# Autodesk Inventor assembly: ktoe
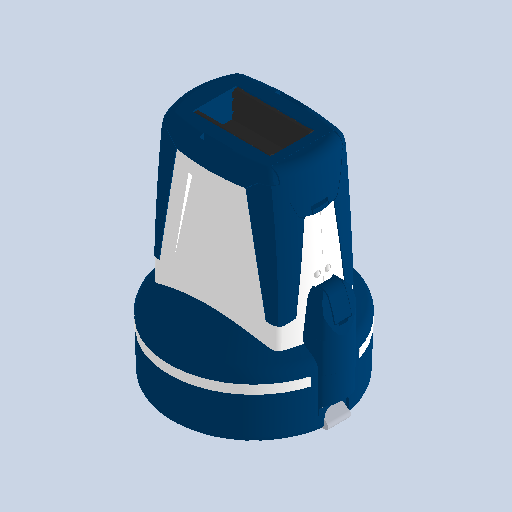
[picture p0: Inventor's stored thumbnail of the model, 512x512]
Saved by Autodesk Inventor 2023 (Build 270158000, 158)
## iProperties
Created: 2022-09-14
Part Number: ktoe
Document SubType Name: Assembly
Designer: Robert
Author: Robert
## Documents named in this file (7)
- C:\Users\Rober\Documents\Ingenieurinformatik\grop\catkin\src\grop\coactegpc\urdf\40\base\ktoe\ktoe.iam
- C:\Users\Rober\Documents\Ingenieurinformatik\grop\catkin\src\grop\coactegpc\urdf\40\base\ktoe\Co-act EGP-C 40 Modell 1.ipt
- C:\Users\Rober\Documents\Ingenieurinformatik\grop\catkin\src\grop\coactegpc\urdf\40\base\ktoe\SCHUNK-1013180-ISO-1-50-M6 Universalflansch Co-act-EGP-C.ipt
- C:\Users\Rober\Documents\Ingenieurinformatik\grop\catkin\src\grop\coactegpc\urdf\40\base\ktoe\SCHUNK-9905502 Typenschild 9x24x0_3.ipt
- C:\Users\Rober\Documents\Ingenieurinformatik\grop\catkin\src\grop\coactegpc\urdf\40\base\ktoe\SCHUNK-5521120 Gehaeuse EGP 40.ipt
- C:\Users\Rober\Documents\Ingenieurinformatik\grop\catkin\src\grop\coactegpc\urdf\40\base\ktoe\SCHUNK-SNT016581 Stecker EGP.ipt
- C:\Users\Rober\Documents\Ingenieurinformatik\grop\catkin\src\grop\coactegpc\urdf\40\base\ktoe\SCHUNK-9700901 Halter fuer NHS Du 4.ipt
## Components (8 placed, 6 different names)
1. Co-act EGP-C 40 Modell 1:1
2. SCHUNK-1013180-ISO-1-50-M6 Universalflansch Co-act-EGP-C:1
3. SCHUNK-9905502 Typenschild 9x24x0_3:1
4. SCHUNK-5521120 Gehaeuse EGP 40:1
5. SCHUNK-SNT016581 Stecker EGP:1
6. SCHUNK-9700901 Halter fuer NHS Du 4:1
7. SCHUNK-9700901 Halter fuer NHS Du 4:2
8. SCHUNK-9905502 Typenschild 9x24x0_3:2
## Relationships (12: Mate 5, Angle 4, Flush 3)
- [Flush]: Co-act EGP-C 40 Modell 1:1 ↔ SCHUNK-1013180-ISO-1-50-M6 Universalflansch Co-act-EGP-C:1
- [Mate]: Co-act EGP-C 40 Modell 1:1 ↔ SCHUNK-1013180-ISO-1-50-M6 Universalflansch Co-act-EGP-C:1
- [Angle] (-30 deg): Co-act EGP-C 40 Modell 1:1 ↔ SCHUNK-1013180-ISO-1-50-M6 Universalflansch Co-act-EGP-C:1
- [Flush] (0.6 mm): Co-act EGP-C 40 Modell 1:1 ↔ SCHUNK-9905502 Typenschild 9x24x0_3:1
- [Mate]: Co-act EGP-C 40 Modell 1:1 ↔ SCHUNK-9905502 Typenschild 9x24x0_3:1
- [Angle] (0 deg): Co-act EGP-C 40 Modell 1:1 ↔ SCHUNK-9905502 Typenschild 9x24x0_3:1
- [Flush]: SCHUNK-5521120 Gehaeuse EGP 40:1 ↔ SCHUNK-9700901 Halter fuer NHS Du 4:1
- [Mate]: SCHUNK-5521120 Gehaeuse EGP 40:1 ↔ SCHUNK-9700901 Halter fuer NHS Du 4:1
- [Angle] (0 deg): SCHUNK-5521120 Gehaeuse EGP 40:1 ↔ SCHUNK-9700901 Halter fuer NHS Du 4:1
- [Mate]: SCHUNK-5521120 Gehaeuse EGP 40:1 ↔ SCHUNK-9905502 Typenschild 9x24x0_3:2
- [Mate]: SCHUNK-5521120 Gehaeuse EGP 40:1 ↔ SCHUNK-9905502 Typenschild 9x24x0_3:2
- [Angle] (0 deg): SCHUNK-5521120 Gehaeuse EGP 40:1 ↔ SCHUNK-9905502 Typenschild 9x24x0_3:2
